# Autodesk Inventor assembly: 217-7263 20200930
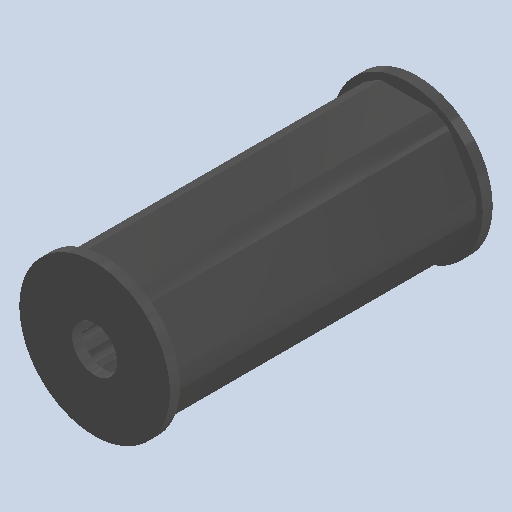
[picture p0: Inventor's stored thumbnail of the model, 512x512]
Saved by Autodesk Inventor 2023.3 (Build 273359000, 359)
## iProperties
Created: 2020-09-30
Part Number: 217-7263 20200930
Description: Falcon Hex Adapter
Document SubType Name: Assembly
Designer: jackc
Sending System: SolidWorks 2019
Preprocessor: SwSTEP 2.0
Title: 217-7263 20200930.STEP
Revision Number: ANY
## Documents named in this file (4)
- D:\.shortcut-targets-by-id\104lhnwPhYvankLacu8RGROV89Bx_24Mg\1939\2_Design\2023-2024\Parts\Motors\Falcon Spline to 1_2 ThunderHex\Falcon Spline to 1_2 ThunderHex Adapter (217-7263).iam
- D:\.shortcut-targets-by-id\104lhnwPhYvankLacu8RGROV89Bx_24Mg\1939\2_Design\2023-2024\Parts\Motors\Falcon Spline to 1_2 ThunderHex\217-7263-001 Rev1.ipt
- D:\.shortcut-targets-by-id\104lhnwPhYvankLacu8RGROV89Bx_24Mg\1939\2_Design\2023-2024\Parts\Motors\Falcon Spline to 1_2 ThunderHex\217-7263-002 Rev2.ipt
- D:\.shortcut-targets-by-id\104lhnwPhYvankLacu8RGROV89Bx_24Mg\1939\2_Design\2023-2024\Parts\Motors\Falcon Spline to 1_2 ThunderHex\217-7263-003 Rev2.ipt
## Components (3 placed, 3 different names)
1. 217-7263-001 Rev1_1 — Mate:1, Mate:2, Mate:4
2. 217-7263-002 Rev2_2 — Mate:2, Mate:3
3. 217-7263-003 Rev2_3 — Mate:1, Mate:3, Mate:4
## Relationships (4: Mate 4)
- Mate:1: 217-7263-001 Rev1_1 ↔ 217-7263-003 Rev2_3
- Mate:2: 217-7263-001 Rev1_1 ↔ 217-7263-002 Rev2_2
- Mate:3: 217-7263-002 Rev2_2 ↔ 217-7263-003 Rev2_3
- Mate:4: 217-7263-001 Rev1_1 ↔ 217-7263-003 Rev2_3
